# Autodesk Inventor assembly: !drive-pod-front-right
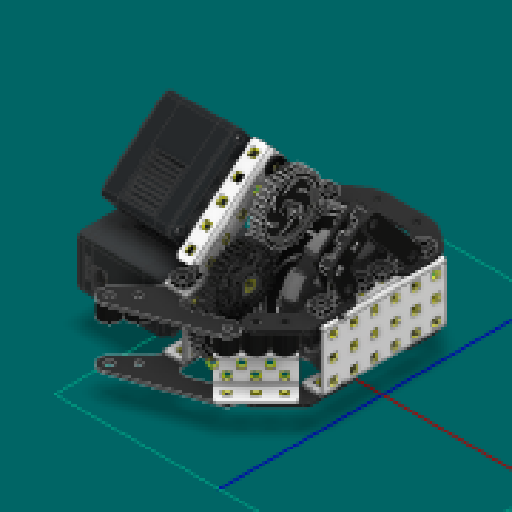
[picture p0: Inventor's stored thumbnail of the model, 512x512]
Saved by Autodesk Inventor 2025 (Build 290162000, 162)
## iProperties
Created: 2024-08-10
Part Number: !drive-pod-front-right
Document SubType Name: Assembly
Designer: averey
Author: averey
## Documents named in this file (24)
- C:\Users\avere\rbp_cad\atlas\chassis\drive-pod-front-right\!drive-pod-front-right.iam
- C:\Users\avere\rbp_cad\atlas\chassis\drive-pod-front-right\Alu C 1x3x1x6-front-right.ipt
- C:\Users\avere\rbp_cad\atlas\chassis\drive-pod-front-right\funnel_gusset-front-right.ipt
- C:\Users\avere\rbp_cad\VEX-CAD-Inventor-1.41\Structure\Standoff\Standoff 1.50.ipt
- C:\Users\avere\rbp_cad\VEX-CAD-Inventor-1.41\Structure\Standoff.ipt
- C:\Users\avere\rbp_cad\atlas\chassis\drive-pod-front-right\LS Pillow Bearing Block-front-right.ipt
- C:\Users\avere\rbp_cad\atlas\chassis\drive-pod-front-right\Alu C 1x3x1x8-front-right.ipt
- C:\Users\avere\rbp_cad\atlas\chassis\drive-pod-front-right\gearbox-support-gusset-front-right.ipt
- C:\Users\avere\rbp_cad\atlas\chassis\drive-pod-front-right\gearbox-gusset-front-right.ipt
- C:\Users\avere\rbp_cad\atlas\chassis\drive-pod-front-right\Bearing Flat Low Profile-front-right.ipt
- C:\Users\avere\rbp_cad\atlas\chassis\drive-pod-front-right\Alu Angle 1x1x5-front-right.ipt
- C:\Users\avere\rbp_cad\atlas\chassis\drive-pod-front-right\SteelM-StarS-front-right.iam
- C:\Users\avere\rbp_cad\atlas\chassis\drive-pod-front-right\V5 Motor (5.5W)-front-right.ipt
- C:\Users\avere\rbp_cad\atlas\chassis\drive-pod-front-right\LS 36T Gear-front-right.ipt
- C:\Users\avere\rbp_cad\atlas\chassis\drive-pod-front-right\LS 60T Gear-front-right.ipt
- C:\Users\avere\rbp_cad\atlas\chassis\drive-pod-front-right\2.75 Omni AS, No Insert-front-right.iam
- C:\Users\avere\rbp_cad\atlas\chassis\drive-pod-front-right\LS 12T Gear-front-right.ipt
- C:\Users\avere\rbp_cad\atlas\chassis\drive-pod-front-right\half_cut_36t-front-right.ipt
- C:\Users\avere\rbp_cad\atlas\chassis\drive-pod-front-right\elbow-gusset-front-right.ipt
- C:\Users\avere\rbp_cad\atlas\chassis\drive-pod-front-right\Alu C 1x2x1x3-front-right.ipt
- C:\Users\avere\rbp_cad\atlas\chassis\drive-pod-front-right\join-gusset_offset-front-right.ipt
- C:\Users\avere\rbp_cad\VEX-CAD-Inventor-1.41\Motion\Spacers\Spacer Nylon .500 OD\NSpacer Black .500 OD x .500.ipt
- C:\Users\avere\rbp_cad\VEX-CAD-Inventor-1.41\Motion\Spacers\Spacer Nylon .500 OD.ipt
- C:\Users\avere\rbp_cad\VEX-CAD-Inventor-1.41\Motion\Spacers\Spacer Nylon .500 OD\NSpacer Black .500 OD x .375.ipt
## Components (36 placed, 21 different names)
1. Alu C 1x3x1x6-front-right:1 — Mate:1, Insert:1, Mate:2, Insert:2, Mate:4, Insert:7, Mate:5, Mate:24, Insert:34, Mate:26, Insert:36
2. funnel_gusset-front-right:1 — Mate:1, Insert:1, Insert:6, Mate:6, Insert:8, Insert:14
3. funnel_gusset-front-right:2 — Mate:2, Insert:2, Insert:4, Insert:5
4. Standoff 1.50:1 — Insert:4
5. Standoff 1.50:2 — Insert:5
6. LS Pillow Bearing Block-front-right:1 — Insert:6, Mate:4, Mate:7, Insert:11
7. LS Pillow Bearing Block-front-right:2 — Insert:7, Mate:5, Insert:9, Mate:8
8. Alu C 1x3x1x8-front-right:1 — Mate:6, Insert:8, Mate:10, Mate:11, Insert:15, Insert:26, Insert:27, Mate:27, Insert:37, Mate:28, Insert:34, Mate:21
9. gearbox-support-gusset-front-right:1 — Insert:9
10. gearbox-gusset-front-right:1 — Mate:7, Mate:9
11. gearbox-support-gusset-front-right:2 — Mate:8
12. gearbox-gusset-front-right:2 — Insert:11
13. Bearing Flat Low Profile-front-right:1 — Mate:9
14. LS Pillow Bearing Block-front-right:3 — Insert:14, Mate:10, Insert:17, Insert:18
15. LS Pillow Bearing Block-front-right:4 — Mate:11, Insert:15, Insert:16
16. Alu Angle 1x1x5-front-right:1 — Insert:16, Mate:12, Mate:13, Mate:22, Insert:31, Insert:30, Insert:32
17. gearbox-gusset-front-right:3 — Mate:12, Insert:17
18. gearbox-gusset-front-right:4 — Mate:13, Insert:18
19. SteelM-StarS-front-right:1 [sub-assembly] — Insert:34, Mate:21
20. V5 Motor (5.5W)-front-right:1 — Mate:22, Insert:31
21. LS 36T Gear-front-right:1 — Insert:26, Insert:29
22. LS 60T Gear-front-right:1 — Insert:27, Insert:28, Mate:21
23. 2.75 Omni AS, No Insert-front-right:1 [sub-assembly] — Insert:28, Mate:21
24. LS 12T Gear-front-right:1 — Insert:29
25. half_cut_36t-front-right:1 — Insert:30
26. LS 36T Gear-front-right:2 — Insert:32
27. elbow-gusset-front-right:1 — Mate:24, Insert:34, Mate:25, Insert:35
28. Alu C 1x2x1x3-front-right:1 — Mate:25, Insert:35, Insert:38, Insert:41
29. elbow-gusset-front-right:2 — Mate:26, Insert:36, Insert:39, Insert:40
30. join-gusset_offset-front-right:1 — Mate:27, Insert:37, Insert:43, Insert:33
31. join-gusset_offset-front-right:2 — Mate:28, Insert:38
32. NSpacer Black .500 OD x .500:1 — Insert:39
33. NSpacer Black .500 OD x .500:2 — Insert:40
34. NSpacer Black .500 OD x .375:3 — Insert:41
35. NSpacer Black .500 OD x .375:4 — Insert:43
36. NSpacer Black .500 OD x .375:5 — Insert:33
## Relationships (52: Insert 32, Mate 20)
- Mate:1: Alu C 1x3x1x6-front-right:1 ↔ funnel_gusset-front-right:1
- Insert:1: Alu C 1x3x1x6-front-right:1 ↔ funnel_gusset-front-right:1
- Mate:2: Alu C 1x3x1x6-front-right:1 ↔ funnel_gusset-front-right:2
- Insert:2: Alu C 1x3x1x6-front-right:1 ↔ funnel_gusset-front-right:2
- Insert:4: funnel_gusset-front-right:2 ↔ Standoff 1.50:1
- Insert:5: funnel_gusset-front-right:2 ↔ Standoff 1.50:2
- Insert:6 (1.5875 mm): funnel_gusset-front-right:1 ↔ LS Pillow Bearing Block-front-right:1
- Mate:4: Alu C 1x3x1x6-front-right:1 ↔ LS Pillow Bearing Block-front-right:1
- Insert:7 (3.175 mm): Alu C 1x3x1x6-front-right:1 ↔ LS Pillow Bearing Block-front-right:2
- Mate:5: Alu C 1x3x1x6-front-right:1 ↔ LS Pillow Bearing Block-front-right:2
- Mate:6: funnel_gusset-front-right:1 ↔ Alu C 1x3x1x8-front-right:1
- Insert:8: funnel_gusset-front-right:1 ↔ Alu C 1x3x1x8-front-right:1
- Insert:9: LS Pillow Bearing Block-front-right:2 ↔ gearbox-support-gusset-front-right:1
- Mate:7: LS Pillow Bearing Block-front-right:1 ↔ gearbox-gusset-front-right:1
- Mate:8: LS Pillow Bearing Block-front-right:2 ↔ gearbox-support-gusset-front-right:2
- Insert:11: LS Pillow Bearing Block-front-right:1 ↔ gearbox-gusset-front-right:2
- Mate:9: gearbox-gusset-front-right:1 ↔ Bearing Flat Low Profile-front-right:1
- Insert:14 (1.5875 mm): funnel_gusset-front-right:1 ↔ LS Pillow Bearing Block-front-right:3
- Mate:10: Alu C 1x3x1x8-front-right:1 ↔ LS Pillow Bearing Block-front-right:3
- Mate:11: Alu C 1x3x1x8-front-right:1 ↔ LS Pillow Bearing Block-front-right:4
- Insert:15: Alu C 1x3x1x8-front-right:1 ↔ LS Pillow Bearing Block-front-right:4
- Insert:16: LS Pillow Bearing Block-front-right:4 ↔ Alu Angle 1x1x5-front-right:1
- Mate:12: Alu Angle 1x1x5-front-right:1 ↔ gearbox-gusset-front-right:3
- Insert:17 (1.5875 mm): LS Pillow Bearing Block-front-right:3 ↔ gearbox-gusset-front-right:3
- Mate:13: Alu Angle 1x1x5-front-right:1 ↔ gearbox-gusset-front-right:4
- Insert:18: LS Pillow Bearing Block-front-right:3 ↔ gearbox-gusset-front-right:4
- Mate:22: Alu Angle 1x1x5-front-right:1 ↔ V5 Motor (5.5W)-front-right:1
- Insert:31: Alu Angle 1x1x5-front-right:1 ↔ V5 Motor (5.5W)-front-right:1
- Insert:26 (0.3969 mm): Alu C 1x3x1x8-front-right:1 ↔ LS 36T Gear-front-right:1
- Insert:27 (0.3969 mm): Alu C 1x3x1x8-front-right:1 ↔ LS 60T Gear-front-right:1
- Insert:28 (19.05 mm): LS 60T Gear-front-right:1 ↔ 2.75 Omni AS, No Insert-front-right:1
- Mate:21: LS 60T Gear-front-right:1 ↔ 2.75 Omni AS, No Insert-front-right:1
- Insert:29: LS 36T Gear-front-right:1 ↔ LS 12T Gear-front-right:1
- Insert:30 (11.5094 mm): Alu Angle 1x1x5-front-right:1 ↔ half_cut_36t-front-right:1
- Insert:32 (12.7 mm): Alu Angle 1x1x5-front-right:1 ↔ LS 36T Gear-front-right:2
- Mate:24: Alu C 1x3x1x6-front-right:1 ↔ elbow-gusset-front-right:1
- Insert:34: Alu C 1x3x1x6-front-right:1 ↔ elbow-gusset-front-right:1
- Mate:25: elbow-gusset-front-right:1 ↔ Alu C 1x2x1x3-front-right:1
- Insert:35: elbow-gusset-front-right:1 ↔ Alu C 1x2x1x3-front-right:1
- Mate:26: Alu C 1x3x1x6-front-right:1 ↔ elbow-gusset-front-right:2
- Insert:36: Alu C 1x3x1x6-front-right:1 ↔ elbow-gusset-front-right:2
- Mate:27: Alu C 1x3x1x8-front-right:1 ↔ join-gusset_offset-front-right:1
- Insert:37: Alu C 1x3x1x8-front-right:1 ↔ join-gusset_offset-front-right:1
- Mate:28: Alu C 1x3x1x8-front-right:1 ↔ join-gusset_offset-front-right:2
- Insert:38: Alu C 1x2x1x3-front-right:1 ↔ join-gusset_offset-front-right:2
- Insert:39: elbow-gusset-front-right:2 ↔ NSpacer Black .500 OD x .500:1
- Insert:40: elbow-gusset-front-right:2 ↔ NSpacer Black .500 OD x .500:2
- Insert:41: Alu C 1x2x1x3-front-right:1 ↔ NSpacer Black .500 OD x .375:3
- Insert:43: join-gusset_offset-front-right:1 ↔ NSpacer Black .500 OD x .375:4
- Insert:33: join-gusset_offset-front-right:1 ↔ NSpacer Black .500 OD x .375:5
- Insert:34: Alu C 1x3x1x8-front-right:1 ↔ SteelM-StarS-front-right:1
- Mate:21: Alu C 1x3x1x8-front-right:1 ↔ SteelM-StarS-front-right:1
